# Autodesk Inventor assembly: Assembly1
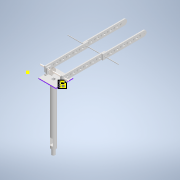
[picture p0: Inventor's stored thumbnail of the model, 180x180]
Saved by Autodesk Inventor 2022 (Build 260153000, 153)
## iProperties
Created: 2022-03-30
Part Number: Assembly1
Document SubType Name: Assembly
Designer: pauly
Author: pauly
## Documents named in this file (11)
- C:\Users\pauly\OneDrive\Documents\Robotics arm\Assembly1.iam
- C:\Users\pauly\OneDrive\Documents\Robotics arm\Shaft connecting chassis updated 1-19.ipt
- C:\Users\pauly\OneDrive\Documents\Robotics arm\base_plate.ipt
- C:\Users\pauly\OneDrive\Documents\Robotics arm\Updated Support_chris.ipt
- C:\Users\pauly\OneDrive\Documents\Robotics arm\am-2986 FR8ZZ Hex Bearing.ipt
- C:\Users\pauly\OneDrive\Documents\Robotics arm\am-0856 500 Hex Shaft for Modulox REV3.ipt
- C:\Users\pauly\OneDrive\Documents\Robotics arm\arm_plate_btw_support_bicep.ipt
- C:\Users\pauly\OneDrive\Documents\Robotics arm\am-4457 8 mm ID 22 mm OD Shielded Flanged Bearing F608ZZ.ipt
- C:\Users\pauly\OneDrive\Documents\Robotics arm\1265K67_Rotary Shaft.ipt
- C:\Users\pauly\OneDrive\Documents\Robotics arm\arm_plate_evan.ipt
- C:\Users\pauly\OneDrive\Documents\Robotics arm\am-3822 56T 20DP 500hex 375 FW.ipt
## Components (15 placed, 10 different names)
1. Shaft connecting chassis updated 1-19:1 — Rotational:1
2. base_plate:1 — Rotational:1, Rotational:2, Rotational:3
3. Updated Support_chris:1 — Rotational:2, Rotational:4, Insert:1
4. Updated Support_chris:2 — Rotational:3, Rotational:5
5. am-2986 FR8ZZ Hex Bearing:1 — Rotational:4, Insert:1
6. am-2986 FR8ZZ Hex Bearing:2 — Rotational:5, Slider:1, Rotational:10
7. am-0856 500 Hex Shaft for Modulox REV3:1 — Slider:1, Slider:2, Slider:3
8. arm_plate_btw_support_bicep:1 — Slider:2, Rotational:7
9. arm_plate_btw_support_bicep:2 — Slider:3, Rotational:6
10. am-4457 8 mm ID 22 mm OD Shielded Flanged Bearing F608ZZ:1 — Rotational:6, Rigid:1
11. am-4457 8 mm ID 22 mm OD Shielded Flanged Bearing F608ZZ:2 — Rotational:7
12. 1265K67_Rotary Shaft:1 — Rigid:1, Rotational:8, Rotational:9
13. arm_plate_evan:1 — Rotational:9
14. arm_plate_evan:2 — Rotational:8
15. am-3822 56T 20DP 500hex 375 FW:1 — Rotational:10
## Relationships (15: RevoluteJoint 10, TranslationJoint 3, Insert 1, WeldJoint 1)
- Rotational:1 [RevoluteJoint]: Shaft connecting chassis updated 1-19:1 ↔ base_plate:1
- Rotational:2 [RevoluteJoint]: base_plate:1 ↔ Updated Support_chris:1
- Rotational:3 [RevoluteJoint]: base_plate:1 ↔ Updated Support_chris:2
- Rotational:4 [RevoluteJoint]: Updated Support_chris:1 ↔ am-2986 FR8ZZ Hex Bearing:1
- Rotational:5 [RevoluteJoint]: Updated Support_chris:2 ↔ am-2986 FR8ZZ Hex Bearing:2
- Insert:1: Updated Support_chris:1 ↔ am-2986 FR8ZZ Hex Bearing:1
- Slider:1 [TranslationJoint]: am-2986 FR8ZZ Hex Bearing:2 ↔ am-0856 500 Hex Shaft for Modulox REV3:1
- Slider:2 [TranslationJoint] (-12.7 mm): am-0856 500 Hex Shaft for Modulox REV3:1 ↔ arm_plate_btw_support_bicep:1
- Slider:3 [TranslationJoint] (-12.7 mm): am-0856 500 Hex Shaft for Modulox REV3:1 ↔ arm_plate_btw_support_bicep:2
- Rotational:6 [RevoluteJoint]: arm_plate_btw_support_bicep:2 ↔ am-4457 8 mm ID 22 mm OD Shielded Flanged Bearing F608ZZ:1
- Rotational:7 [RevoluteJoint] (-3.81 mm): arm_plate_btw_support_bicep:1 ↔ am-4457 8 mm ID 22 mm OD Shielded Flanged Bearing F608ZZ:2
- Rigid:1 [WeldJoint] (-406.4 mm): am-4457 8 mm ID 22 mm OD Shielded Flanged Bearing F608ZZ:1 ↔ 1265K67_Rotary Shaft:1
- Rotational:8 [RevoluteJoint] (-190.5 mm): 1265K67_Rotary Shaft:1 ↔ arm_plate_evan:2
- Rotational:9 [RevoluteJoint] (-165.1 mm): 1265K67_Rotary Shaft:1 ↔ arm_plate_evan:1
- Rotational:10 [RevoluteJoint] (127 mm): am-2986 FR8ZZ Hex Bearing:2 ↔ am-3822 56T 20DP 500hex 375 FW:1
